# Autodesk Inventor assembly: R-W v6
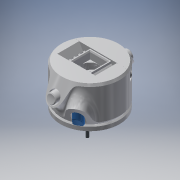
[picture p0: Inventor's stored thumbnail of the model, 180x180]
Saved by Autodesk Inventor 2018.1 (Build 221171000, 171)
## iProperties
Created: 2017-09-22
Part Number: R-W v6
Material: 一般
Document SubType Name: Assembly
Designer: sktom
Author: sktom
## Documents named in this file (13)
- D:\CloudStrage\NextCloud\Cad_mechanical\HACKberry_SizeM\3Dmodel\R\M-R-W\M-R-W.iam
- D:\CloudStrage\NextCloud\Cad_mechanical\HACKberry_SizeM\3Dmodel\R\M-R-W\M-R-W-02.ipt
- D:\CloudStrage\NextCloud\Cad_mechanical\HACKberry_SizeM\3Dmodel\R\M-R-W\M-R-W-01.ipt
- D:\CloudStrage\NextCloud\Cad_mechanical\HACKberry_SizeM\3Dmodel\R\M-R-W\M-R-W-04.ipt
- D:\CloudStrage\NextCloud\Cad_mechanical\HACKberry_SizeM\3Dmodel\R\M-R-W\M-R-W-05.ipt
- D:\CloudStrage\NextCloud\Cad_mechanical\HACKberry_SizeM\3Dmodel\R\M-R-W\M-R-W-06.ipt
- D:\CloudStrage\NextCloud\Cad_mechanical\HACKberry_SizeM\3Dmodel\R\M-R-W\M-R-W-07.ipt
- D:\CloudStrage\NextCloud\Cad_mechanical\HACKberry_SizeM\3Dmodel\R\M-R-W\M-R-W-08.ipt
- D:\CloudStrage\NextCloud\Cad_mechanical\HACKberry_SizeM\3Dmodel\R\M-R-W\M-R-W-03.ipt
- D:\CloudStrage\NextCloud\Cad_mechanical\HACKberry_SizeM\3Dmodel\R\M-R-W\CS 0.29-5.5-8.ipt
- D:\CloudStrage\NextCloud\Cad_mechanical\HACKberry_SizeM\3Dmodel\R\M-R-W\flatScrewM2L6PHI3.3T1.ipt
- D:\CloudStrage\NextCloud\Cad_mechanical\HACKberry_SizeM\3Dmodel\R\M-R-W\ScrewM3L8Btite.ipt
- D:\CloudStrage\NextCloud\Cad_mechanical\HACKberry_SizeM\3Dmodel\R\M-R-W\ScrewM2L10.ipt
## Components (18 placed, 12 different names)
1. R-W-02 v2:1 — リジッド:1, 回転:1, リジッド:3, 回転:4, 回転:5, 回転:6, 円柱状:1, 挿入:1, 挿入:2, 挿入:3
2. R-W-01 v2:1 — リジッド:1
3. R-W-04 v2:1 — 回転:2, 回転:3, 挿入:8, 挿入:9, 挿入:10
4. R-W-05 v2:1 — 回転:1, 回転:2, 回転:3, 挿入:6, 挿入:7
5. R-W-06 v2:1 — リジッド:2
6. R-W-07 v2:1 — リジッド:2, リジッド:3
7. R-W-08 v2:1 — 回転:4, 回転:5, 挿入:4, 挿入:5
8. R-W-03 v1:1 — 回転:6, 円柱状:1
9. CS 0.29-5.5-8:1 — 挿入:1
10. CS 0.29-5.5-8:2 — 挿入:2
11. CS 0.29-5.5-8:3 — 挿入:3
12. ScrewM3L8Btite:1 — 挿入:4
13. ScrewM3L8Btite:2 — 挿入:5
14. flatScrewM2L6PHI3.3T1:1 — 挿入:7
15. flatScrewM2L6PHI3.3T1:2 — 挿入:6
16. ScrewM2L10:1 — 挿入:9
17. ScrewM2L10:2 — 挿入:10
18. ScrewM2L10:3 — 挿入:8
## Relationships (20: Insert 10, RevoluteJoint 6, WeldJoint 3, CylindricalJoint 1)
- リジッド:1 [WeldJoint] (0.5 mm): R-W-02 v2:1 ↔ R-W-01 v2:1
- 回転:1 [RevoluteJoint]: R-W-02 v2:1 ↔ R-W-05 v2:1
- 回転:2 [RevoluteJoint]: R-W-04 v2:1 ↔ R-W-05 v2:1
- 回転:3 [RevoluteJoint]: R-W-04 v2:1 ↔ R-W-05 v2:1
- リジッド:2 [WeldJoint]: R-W-06 v2:1 ↔ R-W-07 v2:1
- リジッド:3 [WeldJoint] (-0.5 mm): R-W-02 v2:1 ↔ R-W-07 v2:1
- 回転:4 [RevoluteJoint]: R-W-02 v2:1 ↔ R-W-08 v2:1
- 回転:5 [RevoluteJoint]: R-W-02 v2:1 ↔ R-W-08 v2:1
- 回転:6 [RevoluteJoint] (2 mm): R-W-02 v2:1 ↔ R-W-03 v1:1
- 円柱状:1 [CylindricalJoint]: R-W-02 v2:1 ↔ R-W-03 v1:1
- 挿入:1 [Insert]: R-W-02 v2:1 ↔ CS 0.29-5.5-8:1
- 挿入:2 [Insert]: R-W-02 v2:1 ↔ CS 0.29-5.5-8:2
- 挿入:3 [Insert]: R-W-02 v2:1 ↔ CS 0.29-5.5-8:3
- 挿入:4 [Insert]: R-W-08 v2:1 ↔ ScrewM3L8Btite:1
- 挿入:5 [Insert]: R-W-08 v2:1 ↔ ScrewM3L8Btite:2
- 挿入:6 [Insert]: R-W-05 v2:1 ↔ flatScrewM2L6PHI3.3T1:2
- 挿入:7 [Insert]: R-W-05 v2:1 ↔ flatScrewM2L6PHI3.3T1:1
- 挿入:8 [Insert]: R-W-04 v2:1 ↔ ScrewM2L10:3
- 挿入:9 [Insert]: R-W-04 v2:1 ↔ ScrewM2L10:1
- 挿入:10 [Insert]: R-W-04 v2:1 ↔ ScrewM2L10:2
